# Autodesk Inventor assembly: Module with Cover V1
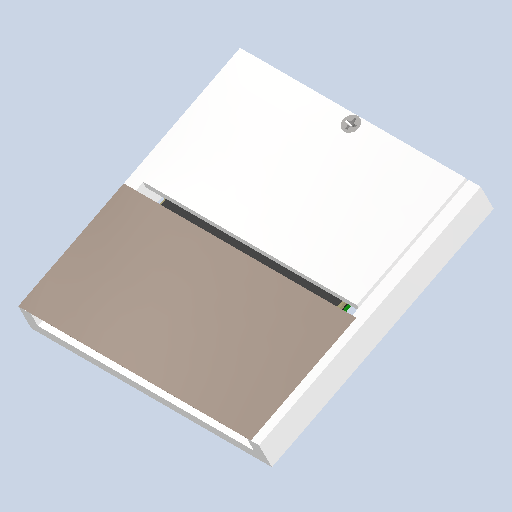
[picture p0: Inventor's stored thumbnail of the model, 512x512]
Saved by Autodesk Inventor 2025 (Build 290162000, 162)
## iProperties
Created: 2024-03-28
Part Number: Module with Cover V1
Document SubType Name: Assembly
Designer: cfang
Author: cfang
## Documents named in this file (7)
- C:\Users\cfang\Desktop\nebraska-silicon-lab\Hardware\ETL\Irradiation Fixture\Module with Cover V1.iam
- C:\Users\cfang\Desktop\nebraska-silicon-lab\Hardware\ETL\modules\tamale v1.5\Tamale - V1p5p2.iam
- C:\Users\cfang\Desktop\nebraska-silicon-lab\Hardware\ETL\Irradiation Fixture\Module Holder V1.ipt
- C:\Users\cfang\Desktop\nebraska-silicon-lab\Hardware\ETL\Irradiation Fixture\Glass Slide Spacer V1.ipt
- C:\Users\cfang\Desktop\nebraska-silicon-lab\Hardware\ETL\Irradiation Fixture\Module Holder Cover V1.ipt
- C:\Users\cfang\Desktop\nebraska-silicon-lab\Hardware\ETL\Irradiation Fixture\Kapton Cover.ipt
- C:\Users\cfang\Desktop\nebraska-silicon-lab\Hardware\ETL\Irradiation Fixture\91420A003_Steel Phillips Flat Head Screws\91420A003_Steel Phillips Flat Head Screws.ipt
## Components (6 placed, 6 different names)
1. Tamale - V1p5p2:1 [sub-assembly] — Insert:2
2. Module Holder V1:1 — Insert:2
3. Glass Slide Spacer V1:1
4. Module Holder Cover V1:1 — Insert:1
5. Kapton Cover:1
6. 91420A003_Steel Phillips Flat Head Screws:1 — Insert:1
## Relationships (11: Mate 6, Flush 3, Insert 2)
- [Mate]: Tamale - V1p5p2:1 ↔ Module Holder V1:1
- [Mate]: Tamale - V1p5p2:1 ↔ Glass Slide Spacer V1:1
- [Flush]: Tamale - V1p5p2:1 ↔ Glass Slide Spacer V1:1
- [Mate] (0.6 mm): Tamale - V1p5p2:1 ↔ Glass Slide Spacer V1:1
- [Mate]: Tamale - V1p5p2:1 ↔ Module Holder Cover V1:1
- [Mate] (0.25 mm): Module Holder V1:1 ↔ Module Holder Cover V1:1
- [Mate]: Module Holder V1:1 ↔ Kapton Cover:1
- [Flush]: Module Holder V1:1 ↔ Kapton Cover:1
- [Flush]: Module Holder V1:1 ↔ Kapton Cover:1
- Insert:1 (-0.254 mm): Module Holder Cover V1:1 ↔ 91420A003_Steel Phillips Flat Head Screws:1
- Insert:2: Tamale - V1p5p2:1 ↔ Module Holder V1:1
## Named parameters: d3_d5 = 0.6 mm, d4_d6 = 0 mm, d5_d7 = 0.25 mm
